# Autodesk Inventor assembly: 000.005.004 - Поворот сгиба кисти СБ
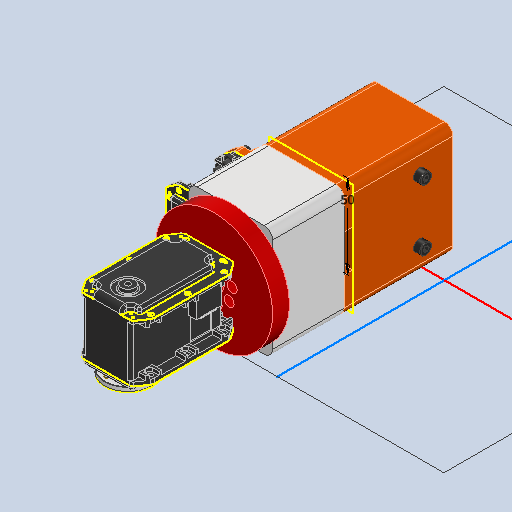
[picture p0: Inventor's stored thumbnail of the model, 512x512]
Saved by Autodesk Inventor 2022 (Build 260153000, 153)
## iProperties
Created: 2022-12-17
Part Number: 000.005.004 - Поворот сгиба кисти СБ
Document SubType Name: Assembly
Designer: Petrov Ivan
Mass: 309.284 g
Surface Area: 856.638 cm^2
Volume: 287.74 cm^3
Density: 1.07487 g/cm^3
Author: Petrov Ivan
## Documents named in this file (12)
- D:\IVAN\Ivan_desktop\Kvantorium\Projects\YouBotRobot\design\000.005.004 - Поворот сгиба кисти СБ.iam
- D:\IVAN\Ivan_desktop\Kvantorium\Projects\YouBotRobot\design\000.005.004.001 - Основание.ipt
- D:\IVAN\Ivan_desktop\Kvantorium\Projects\YouBotRobot\design\standart_components\dynamixels\mx-64\MX-64T.iam
- D:\IVAN\Ivan_desktop\Kvantorium\Projects\YouBotRobot\design\Content Center Files\R2022\ru-RU\BS EN 24035\ISO 4035 - M2.5BS EN.ipt
- D:\IVAN\Ivan_desktop\Kvantorium\Projects\YouBotRobot\design\Content Center Files\R2022\ru-RU\ISO 4762(1)\DIN EN ISO 4762 - M2.5 x 12.ipt
- D:\IVAN\Ivan_desktop\Kvantorium\Projects\YouBotRobot\design\Content Center Files\R2022\ru-RU\ISO 4762(1)\DIN EN ISO 4762 - M2.5 x 25.ipt
- D:\IVAN\Ivan_desktop\Kvantorium\Projects\YouBotRobot\design\000.005.004.002 - Скоба.ipt
- D:\IVAN\Ivan_desktop\Kvantorium\Projects\YouBotRobot\design\Content Center Files\R2022\ru-RU\ISO 4762(1)\DIN EN ISO 4762 - M2.5 x 10.ipt
- D:\IVAN\Ivan_desktop\Kvantorium\Projects\YouBotRobot\design\000.005.004.003 - Поворотный диск.ipt
- D:\IVAN\Ivan_desktop\Kvantorium\Projects\YouBotRobot\design\Content Center Files\R2022\ru-RU\ISO 4762(1)\DIN EN ISO 4762 - M2.5 x 6.ipt
- D:\IVAN\Ivan_desktop\Kvantorium\Projects\YouBotRobot\design\Content Center Files\R2022\ru-RU\ISO 4762(1)\DIN EN ISO 4762 - M4 x 16.ipt
- D:\IVAN\Ivan_desktop\Kvantorium\Projects\YouBotRobot\design\Content Center Files\R2022\ru-RU\ISO 4762(1)\DIN EN ISO 4762 - M2.5 x 16.ipt
## Components (37 placed, 11 different names)
1. 000.005.004.001 - Основание:1 — Угол:3, Совмещение:5, Совмещение:6, Вставка:9, Вставка:10, Вставка:11, Вставка:12, Вставка:14, Вставка:15, Заподлицо:1, Заподлицо:2, Совмещение:13, Вставка:29, Вставка:30, Вставка:31, Вставка:32, Вставка:33, Вставка:34
2. MX-64T:1 [sub-assembly] — Угол:3, Совмещение:5, Совмещение:6, Вставка:1, Вставка:2, Вставка:3, Вставка:4, Вставка:5, Вставка:6, Вставка:7, Вставка:8, Совмещение:9, Совмещение:10, Совмещение:11
3. 000.005.004.002 - Скоба:1 — Заподлицо:1, Заподлицо:2, Вставка:17, Вставка:18, Вставка:19, Вставка:20, Совмещение:13
4. 000.005.004.003 - Поворотный диск:1 — Совмещение:9, Совмещение:10, Совмещение:11, Вставка:21, Вставка:22, Вставка:23, Вставка:24, Вставка:25, Вставка:26, Вставка:27, Вставка:28, Совмещение:12
5. MX-64T:2 [sub-assembly] — Совмещение:12
6. DIN EN ISO 4762 M4 x 16:1 — Вставка:29
7. DIN EN ISO 4762 M4 x 16:2 — Вставка:30
8. DIN EN ISO 4762 M4 x 16:3 — Вставка:31
9. DIN EN ISO 4762 M4 x 16:4 — Вставка:32
10. DIN EN ISO 4762 M2,5 x 16:1 — Вставка:33
11. DIN EN ISO 4762 M2,5 x 16:2 — Вставка:34
12. DIN EN ISO 4762 M2,5 x 10:1 — Вставка:17
13. DIN EN ISO 4762 M2,5 x 10:2 — Вставка:18
14. DIN EN ISO 4762 M2,5 x 10:3 — Вставка:19
15. DIN EN ISO 4762 M2,5 x 10:4 — Вставка:20
16. BS EN 24035 - метрическая M2,5:1 — Вставка:1
17. BS EN 24035 - метрическая M2,5:2 — Вставка:2
18. BS EN 24035 - метрическая M2,5:3 — Вставка:3
19. BS EN 24035 - метрическая M2,5:4 — Вставка:4
20. BS EN 24035 - метрическая M2,5:5 — Вставка:5
21. BS EN 24035 - метрическая M2,5:6 — Вставка:6
22. BS EN 24035 - метрическая M2,5:7 — Вставка:7
23. BS EN 24035 - метрическая M2,5:8 — Вставка:8
24. DIN EN ISO 4762 M2,5 x 12:1 — Вставка:9
25. DIN EN ISO 4762 M2,5 x 12:2 — Вставка:10
26. DIN EN ISO 4762 M2,5 x 12:3 — Вставка:11
27. DIN EN ISO 4762 M2,5 x 12:4 — Вставка:12
28. DIN EN ISO 4762 M2,5 x 25:2 — Вставка:14
29. DIN EN ISO 4762 M2,5 x 25:3 — Вставка:15
30. DIN EN ISO 4762 M2,5 x 6:1 — Вставка:21
31. DIN EN ISO 4762 M2,5 x 6:2 — Вставка:22
32. DIN EN ISO 4762 M2,5 x 6:3 — Вставка:23
33. DIN EN ISO 4762 M2,5 x 6:4 — Вставка:24
34. DIN EN ISO 4762 M2,5 x 6:5 — Вставка:25
35. DIN EN ISO 4762 M2,5 x 6:6 — Вставка:26
36. DIN EN ISO 4762 M2,5 x 6:7 — Вставка:27
37. DIN EN ISO 4762 M2,5 x 6:8 — Вставка:28
## Relationships (42: Insert 32, Mate 7, Flush 2, Angle 1)
- Угол:3 [Angle] (-90 deg): 000.005.004.001 - Основание:1 ↔ MX-64T:1
- Совмещение:5 [Mate]: 000.005.004.001 - Основание:1 ↔ MX-64T:1
- Совмещение:6 [Mate]: 000.005.004.001 - Основание:1 ↔ MX-64T:1
- Вставка:1 [Insert]: MX-64T:1 ↔ BS EN 24035 - метрическая M2,5:1
- Вставка:2 [Insert]: MX-64T:1 ↔ BS EN 24035 - метрическая M2,5:2
- Вставка:3 [Insert]: MX-64T:1 ↔ BS EN 24035 - метрическая M2,5:3
- Вставка:4 [Insert]: MX-64T:1 ↔ BS EN 24035 - метрическая M2,5:4
- Вставка:5 [Insert]: MX-64T:1 ↔ BS EN 24035 - метрическая M2,5:5
- Вставка:6 [Insert]: MX-64T:1 ↔ BS EN 24035 - метрическая M2,5:6
- Вставка:7 [Insert]: MX-64T:1 ↔ BS EN 24035 - метрическая M2,5:7
- Вставка:8 [Insert]: MX-64T:1 ↔ BS EN 24035 - метрическая M2,5:8
- Вставка:9 [Insert]: 000.005.004.001 - Основание:1 ↔ DIN EN ISO 4762 M2,5 x 12:1
- Вставка:10 [Insert]: 000.005.004.001 - Основание:1 ↔ DIN EN ISO 4762 M2,5 x 12:2
- Вставка:11 [Insert]: 000.005.004.001 - Основание:1 ↔ DIN EN ISO 4762 M2,5 x 12:3
- Вставка:12 [Insert]: 000.005.004.001 - Основание:1 ↔ DIN EN ISO 4762 M2,5 x 12:4
- Вставка:14 [Insert]: 000.005.004.001 - Основание:1 ↔ DIN EN ISO 4762 M2,5 x 25:2
- Вставка:15 [Insert]: 000.005.004.001 - Основание:1 ↔ DIN EN ISO 4762 M2,5 x 25:3
- Заподлицо:1 [Flush]: 000.005.004.001 - Основание:1 ↔ 000.005.004.002 - Скоба:1
- Заподлицо:2 [Flush]: 000.005.004.001 - Основание:1 ↔ 000.005.004.002 - Скоба:1
- Вставка:17 [Insert]: 000.005.004.002 - Скоба:1 ↔ DIN EN ISO 4762 M2,5 x 10:1
- Вставка:18 [Insert]: 000.005.004.002 - Скоба:1 ↔ DIN EN ISO 4762 M2,5 x 10:2
- Вставка:19 [Insert]: 000.005.004.002 - Скоба:1 ↔ DIN EN ISO 4762 M2,5 x 10:3
- Вставка:20 [Insert]: 000.005.004.002 - Скоба:1 ↔ DIN EN ISO 4762 M2,5 x 10:4
- Совмещение:9 [Mate]: MX-64T:1 ↔ 000.005.004.003 - Поворотный диск:1
- Совмещение:10 [Mate]: MX-64T:1 ↔ 000.005.004.003 - Поворотный диск:1
- Совмещение:11 [Mate]: MX-64T:1 ↔ 000.005.004.003 - Поворотный диск:1
- Вставка:21 [Insert]: 000.005.004.003 - Поворотный диск:1 ↔ DIN EN ISO 4762 M2,5 x 6:1
- Вставка:22 [Insert]: 000.005.004.003 - Поворотный диск:1 ↔ DIN EN ISO 4762 M2,5 x 6:2
- Вставка:23 [Insert]: 000.005.004.003 - Поворотный диск:1 ↔ DIN EN ISO 4762 M2,5 x 6:3
- Вставка:24 [Insert]: 000.005.004.003 - Поворотный диск:1 ↔ DIN EN ISO 4762 M2,5 x 6:4
- Вставка:25 [Insert]: 000.005.004.003 - Поворотный диск:1 ↔ DIN EN ISO 4762 M2,5 x 6:5
- Вставка:26 [Insert]: 000.005.004.003 - Поворотный диск:1 ↔ DIN EN ISO 4762 M2,5 x 6:6
- Вставка:27 [Insert]: 000.005.004.003 - Поворотный диск:1 ↔ DIN EN ISO 4762 M2,5 x 6:7
- Вставка:28 [Insert]: 000.005.004.003 - Поворотный диск:1 ↔ DIN EN ISO 4762 M2,5 x 6:8
- Совмещение:12 [Mate]: 000.005.004.003 - Поворотный диск:1 ↔ MX-64T:2
- Совмещение:13 [Mate]: 000.005.004.001 - Основание:1 ↔ 000.005.004.002 - Скоба:1
- Вставка:29 [Insert]: 000.005.004.001 - Основание:1 ↔ DIN EN ISO 4762 M4 x 16:1
- Вставка:30 [Insert]: 000.005.004.001 - Основание:1 ↔ DIN EN ISO 4762 M4 x 16:2
- Вставка:31 [Insert]: 000.005.004.001 - Основание:1 ↔ DIN EN ISO 4762 M4 x 16:3
- Вставка:32 [Insert]: 000.005.004.001 - Основание:1 ↔ DIN EN ISO 4762 M4 x 16:4
- Вставка:33 [Insert]: 000.005.004.001 - Основание:1 ↔ DIN EN ISO 4762 M2,5 x 16:1
- Вставка:34 [Insert]: 000.005.004.001 - Основание:1 ↔ DIN EN ISO 4762 M2,5 x 16:2
